# Autodesk Inventor assembly: Bed
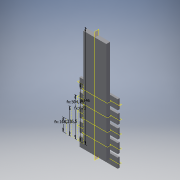
[picture p0: Inventor's stored thumbnail of the model, 180x180]
Saved by Autodesk Inventor 2017 (Build 210142000, 142)
## iProperties
Created: 2019-07-06
Part Number: Bed
Document SubType Name: Assembly
Designer: Ole Simmering
Author: Ole Simmering
## Documents named in this file (3)
- C:\Users\Ole Simmering\Documents\GitHub\3D_modeling\Guillotine\Bed.iam
- C:\Users\Ole Simmering\Documents\GitHub\3D_modeling\Guillotine\BedPlate.ipt
- C:\Users\Ole Simmering\Documents\GitHub\3D_modeling\Guillotine\BedBoard.ipt
## Components (6 placed, 2 different names)
1. BedPlate:1 — Mate:1, Mate:2, Flush:1, Flush:2, Flush:3, Flush:4, Mate:4, Flush:6, Flush:8, Mate:5, Flush:9, Flush:12, Mate:6
2. BedBoard:1 — Mate:1, Mate:2, Mate:3
3. BedBoard:2 — Mate:4, Flush:5, Flush:6
4. BedBoard:3 — Flush:7, Flush:8, Mate:5, Flush:11
5. BedBoard:4 — Flush:9, Flush:10, Flush:11, Flush:13
6. BedBoard:5 — Flush:12, Flush:13, Mate:6
## Relationships (19: Flush 13, Mate 6)
- Mate:1: BedPlate:1 ↔ BedBoard:1
- Mate:2: BedPlate:1 ↔ BedBoard:1
- Flush:1 (-673 mm): BedPlate:1
- Flush:2 (-504.75 mm): BedPlate:1
- Flush:3 (-336.5 mm): BedPlate:1
- Flush:4 (-168.25 mm): BedPlate:1
- Mate:3: BedBoard:1
- Mate:4: BedPlate:1 ↔ BedBoard:2
- Flush:5: BedBoard:2
- Flush:6: BedPlate:1 ↔ BedBoard:2
- Flush:7: BedBoard:3
- Flush:8: BedPlate:1 ↔ BedBoard:3
- Mate:5: BedPlate:1 ↔ BedBoard:3
- Flush:9: BedPlate:1 ↔ BedBoard:4
- Flush:10: BedBoard:4
- Flush:11: BedBoard:3 ↔ BedBoard:4
- Flush:12: BedPlate:1 ↔ BedBoard:5
- Flush:13: BedBoard:4 ↔ BedBoard:5
- Mate:6: BedPlate:1 ↔ BedBoard:5
